# Autodesk Inventor assembly: Kraftübertragung mit Keilriemen
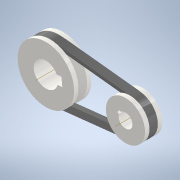
[picture p0: Inventor's stored thumbnail of the model, 180x180]
Saved by Autodesk Inventor 2021 (Build 250183000, 183)
## iProperties
ClientObjectVersion: 1
Created: 2021-01-13
Part Number: Kraftübertragung mit Keilriemen
Document SubType Name: Assembly
Designer: Jaro Machnow
Author: Jaro Machnow
## Documents named in this file (4)
- C:\Users\Jaro Machnow\Documents\Vault\Gruppen\Gruppe 2\Entwurf\Amphibienfahrzeug\Wechsel zwischen Land und Wasser\Wechselmechanik\Klappmechanismus\OldVersions\Kraftübertragung mit Keilriemen.iam
- C:\Users\Jaro Machnow\Desktop\JARO\UNI\Konstruktion\3. Semester\Amphibienfahrzeug\Klapp-Baugruppe\Konstruktions-Assistent\Keilriemen2.ipt
- C:\Users\Jaro Machnow\Desktop\JARO\UNI\Konstruktion\3. Semester\Amphibienfahrzeug\Klapp-Baugruppe\Konstruktions-Assistent\Keilriemenscheibe12.ipt
- C:\Users\Jaro Machnow\Desktop\JARO\UNI\Konstruktion\3. Semester\Amphibienfahrzeug\Klapp-Baugruppe\Konstruktions-Assistent\Keilriemenscheibe22.ipt
## Components (3 placed, 3 different names)
1. Keilriemenscheibe1:1 — Fluchtend:1, Passend:1, Drehung:1
2. Keilriemenscheibe2:1 — Fluchtend:2, Passend:2, Drehung:1
3. Keilriemen:1 — Fluchtend:1, Passend:1, Fluchtend:2, Passend:2
## Component patterns: (1 elements, first: Keilriemen:1)
## Relationships (5: Flush 2, Mate 2, RelateRotation 1)
- Fluchtend:1 [Flush]: Keilriemenscheibe1:1 ↔ Keilriemen:1
- Passend:1 [Mate]: Keilriemenscheibe1:1 ↔ Keilriemen:1
- Fluchtend:2 [Flush]: Keilriemenscheibe2:1 ↔ Keilriemen:1
- Passend:2 [Mate]: Keilriemenscheibe2:1 ↔ Keilriemen:1
- Drehung:1 [RelateRotation] (0.6667 ul): Keilriemenscheibe1:1 ↔ Keilriemenscheibe2:1
